# Autodesk Inventor assembly: Clamp with Piston Assembly
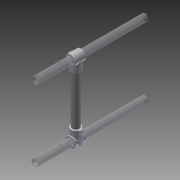
[picture p0: Inventor's stored thumbnail of the model, 180x180]
Saved by Autodesk Inventor 2014 SP1 (Build 180222100, 222)
## iProperties
Created: 2014-01-12
Part Number: Clamp with Piston Assembly
Document SubType Name: Assembly
Designer: Michael
Mass: 305.276 g
Surface Area: 1793.78 cm^2
Volume: 181.752 cm^3
Density: 1.67964 g/cm^3
Author: Michael
## Documents named in this file (4)
- C:\Users\Arpan\Documents\GitHub\2014buildCAD\Collector\Clamp with Piston Assembly.iam
- C:\Users\Arpan\Documents\GitHub\2014buildCAD\Collector\Polycarbonate Clamp Tube (Middle) (8585K14).ipt
- C:\Users\Arpan\Documents\GitHub\2014buildCAD\Collector\Polycarbonate Clamp Tube 1 in OD (8585K14).ipt
- C:\Users\Arpan\Documents\GitHub\2014buildCAD\Collector\Metal Pipe T Joint (4698T140).ipt
## Components (5 placed, 3 different names)
1. Polycarbonate Clamp Tube (Middle) (8585K14):1 — Mate:12, Mate:13
2. Polycarbonate Clamp Tube 1 in OD (8585K14):1 — Angle:1, Mate:10, Mate:11, Mate:16
3. Polycarbonate Clamp Tube 1 in OD (8585K14):2 — Angle:1, Mate:9, Flush:1, Mate:16
4. Metal Pipe T Joint (4698T140):1 — Mate:9, Flush:1, Mate:13, Mate:17
5. Metal Pipe T Joint (4698T140):2 — Mate:10, Mate:11, Mate:12, Mate:17
## Relationships (9: Mate 7, Angle 1, Flush 1)
- Angle:1 (0 deg): Polycarbonate Clamp Tube 1 in OD (8585K14):1 ↔ Polycarbonate Clamp Tube 1 in OD (8585K14):2
- Mate:9: Polycarbonate Clamp Tube 1 in OD (8585K14):2 ↔ Metal Pipe T Joint (4698T140):1
- Mate:10: Polycarbonate Clamp Tube 1 in OD (8585K14):1 ↔ Metal Pipe T Joint (4698T140):2
- Mate:11 (127 mm): Polycarbonate Clamp Tube 1 in OD (8585K14):1 ↔ Metal Pipe T Joint (4698T140):2
- Mate:12: Polycarbonate Clamp Tube (Middle) (8585K14):1 ↔ Metal Pipe T Joint (4698T140):2
- Flush:1 (127 mm): Polycarbonate Clamp Tube 1 in OD (8585K14):2 ↔ Metal Pipe T Joint (4698T140):1
- Mate:13: Polycarbonate Clamp Tube (Middle) (8585K14):1 ↔ Metal Pipe T Joint (4698T140):1
- Mate:16: Polycarbonate Clamp Tube 1 in OD (8585K14):1 ↔ Polycarbonate Clamp Tube 1 in OD (8585K14):2
- Mate:17 (176.276 mm): Metal Pipe T Joint (4698T140):1 ↔ Metal Pipe T Joint (4698T140):2
